# Autodesk Inventor assembly: FinalShooterStorage-ver1-1111-2021
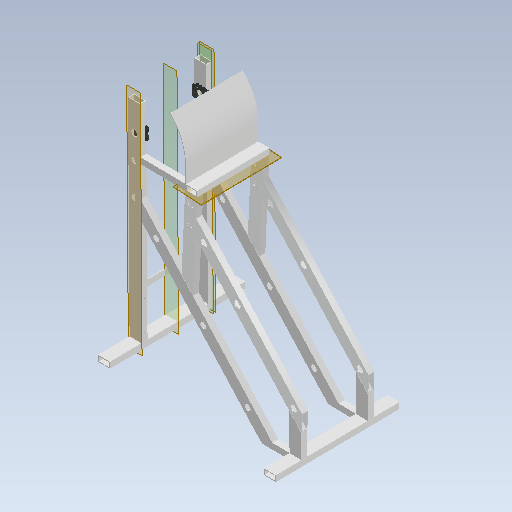
[picture p0: Inventor's stored thumbnail of the model, 512x512]
Saved by Autodesk Inventor 2021 (Build 250183000, 183)
## iProperties
Created: 2021-03-18
Part Number: FinalShooterStorage-ver1-1111-2021
Document SubType Name: Assembly
Designer: CMurray
Author: CMurray
## Documents named in this file (3)
- C:\Users\CMurray\OneDrive\Documents\GitHub\RoboticsCad1111\PHRC CADD\2020 Infinite Recharge\Storage\Assemblies\FinalShooterStorage-ver1-1111-2021.iam
- C:\Users\CMurray\OneDrive\Documents\GitHub\RoboticsCad1111\PHRC CADD\2020 Infinite Recharge\Shooting\Assemblies\ShooterPrototype-ver3-1111-2021.iam
- C:\Users\CMurray\OneDrive\Documents\GitHub\RoboticsCad1111\PHRC CADD\2020 Infinite Recharge\Storage\Assemblies\StorageAssembly-ver5-1111-2021.iam
## Components (2 placed, 2 different names)
1. ShooterPrototype-ver3-1111-2021:1 [sub-assembly] — Mate:1, Flush:1
2. StorageAssembly-ver5-1111-2021:1 [sub-assembly] — Mate:1, Flush:1
## Relationships (2: Mate 1, Flush 1)
- Mate:1: ShooterPrototype-ver3-1111-2021:1 ↔ StorageAssembly-ver5-1111-2021:1
- Flush:1: ShooterPrototype-ver3-1111-2021:1 ↔ StorageAssembly-ver5-1111-2021:1
